# Autodesk Inventor assembly: Сборка1
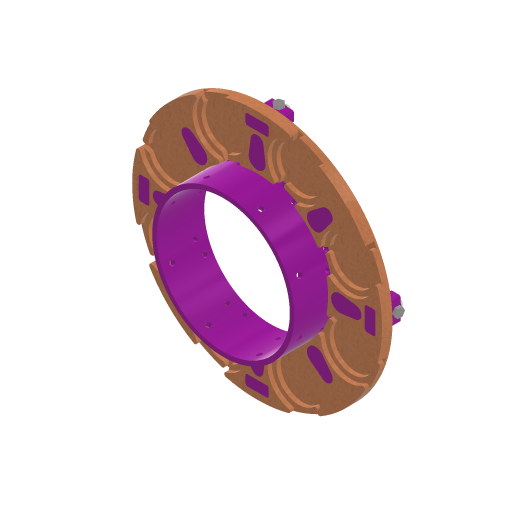
[picture p0: Inventor's stored thumbnail of the model, 512x512]
Saved by Autodesk Inventor 2023 (Build 270158000, 158)
## iProperties
Created: 2023-03-21
Part Number: Сборка1
Document SubType Name: Assembly
Designer: Admin
Author: Admin
## Documents named in this file (9)
- C:\Users\aleks\OneDrive\Рабочий стол\Хроматографический сортировщик\Детали\Хроматографичекий сортировщик.iam
- C:\Users\aleks\OneDrive\Рабочий стол\Хроматографический сортировщик\Детали\Барабан.ipt
- C:\Users\aleks\OneDrive\Рабочий стол\Хроматографический сортировщик\Детали\Покупные\Подшипник.ipt
- C:\Users\aleks\OneDrive\Рабочий стол\Хроматографический сортировщик\Детали\Покупные\Болт М5.ipt
- C:\Users\aleks\OneDrive\Рабочий стол\Хроматографический сортировщик\Детали\Покупные\Гайка М5 стопорная.ipt
- C:\Users\aleks\OneDrive\Рабочий стол\Хроматографический сортировщик\Детали\Покупные\Магнит.ipt
- C:\Users\aleks\OneDrive\Рабочий стол\Хроматографический сортировщик\Детали\Капсуль.ipt
- C:\Users\aleks\OneDrive\Рабочий стол\Хроматографический сортировщик\Детали\Покупные\Болт М5 круглый.ipt
- C:\Users\aleks\OneDrive\Рабочий стол\Хроматографический сортировщик\Детали\Короб для подшипника 2.0.ipt
## Components (49 placed, 8 different names)
1. Барабан:1 — Совмещение:57, Совмещение:58, Заподлицо:13, Совмещение:62, Совмещение:63, Совмещение:68, Совмещение:69, Заподлицо:15, Совмещение:70, Совмещение:71, Совмещение:76, Совмещение:77, Заподлицо:16, Совмещение:78, Совмещение:79, Заподлицо:17, Совмещение:84, Совмещение:85, Совмещение:102, Заподлицо:18, Совмещение:103, Совмещение:104, Заподлицо:19, Совмещение:105, Совмещение:106, Совмещение:107, Заподлицо:20, Совмещение:108, Совмещение:109, Заподлицо:21, Совмещение:111, Совмещение:112, Совмещение:113, Совмещение:114, Совмещение:115, Совмещение:116, Совмещение:117, Совмещение:118, Совмещение:119, Заподлицо:22, Совмещение:126, Совмещение:127, Заподлицо:23, Совмещение:134, Совмещение:135, Заподлицо:24, Совмещение:142, Совмещение:143, Заподлицо:25, Совмещение:150, Совмещение:151
2. Подшипник:1 — Совмещение:136, Совмещение:141
3. Подшипник:2 — Совмещение:128, Совмещение:131
4. Подшипник:3 — Совмещение:121, Совмещение:124
5. Подшипник:4 — Совмещение:145, Совмещение:146, Совмещение:148
6. Болт М5:1 — Совмещение:128, Совмещение:129, Совмещение:130, Совмещение:133
7. Гайка М5 стопорная:1 — Совмещение:129, Совмещение:132
8. Болт М5:2 — Совмещение:136, Совмещение:137, Совмещение:138, Совмещение:140
9. Гайка М5 стопорная:2 — Совмещение:137, Совмещение:139
10. Болт М5:3 — Совмещение:144, Совмещение:146, Совмещение:149
11. Гайка М5 стопорная:3 — Совмещение:122, Совмещение:123
12. Болт М5:4 — Совмещение:120, Совмещение:121, Совмещение:125
13. Гайка М5 стопорная:4 — Совмещение:145, Совмещение:147
14. Магнит:1 — Совмещение:94, Совмещение:95
15. Магнит:2 — Совмещение:66, Совмещение:67
16. Магнит:3 — Совмещение:59, Заподлицо:14
17. Магнит:4 — Совмещение:88, Совмещение:89
18. Магнит:5 — Совмещение:90, Совмещение:91
19. Магнит:6 — Совмещение:82, Совмещение:83
20. Магнит:7 — Совмещение:100, Совмещение:101
21. Магнит:8 — Совмещение:72, Совмещение:73
22. Капсуль:1 — Совмещение:57, Совмещение:58, Заподлицо:13, Совмещение:59, Заподлицо:14, Совмещение:60, Совмещение:61, Угол:1
23. Гайка М5 стопорная:5 — Совмещение:60, Совмещение:61, Угол:1
24. Болт М5 круглый:1 — Совмещение:62, Совмещение:63
25. Капсуль:2 — Совмещение:64, Угол:2, Совмещение:65, Совмещение:66, Совмещение:67, Совмещение:68, Совмещение:69, Заподлицо:15
26. Капсуль:3 — Совмещение:90, Совмещение:91, Совмещение:92, Угол:6, Совмещение:93, Совмещение:108, Совмещение:109, Заподлицо:21
27. Капсуль:4 — Совмещение:72, Совмещение:73, Совмещение:74, Угол:3, Совмещение:75, Совмещение:76, Совмещение:77, Заподлицо:16
28. Капсуль:5 — Совмещение:80, Угол:4, Совмещение:81, Совмещение:82, Совмещение:83, Заподлицо:17, Совмещение:84, Совмещение:85
29. Капсуль:6 — Совмещение:86, Угол:5, Совмещение:87, Совмещение:88, Совмещение:89, Совмещение:102, Заподлицо:18, Совмещение:103
30. Капсуль:7 — Совмещение:94, Совмещение:95, Совмещение:96, Угол:7, Совмещение:97, Совмещение:104, Заподлицо:19, Совмещение:105
31. Капсуль:8 — Совмещение:98, Угол:8, Совмещение:99, Совмещение:100, Совмещение:101, Совмещение:106, Совмещение:107, Заподлицо:20
32. Болт М5 круглый:2 — Совмещение:114, Совмещение:115
33. Гайка М5 стопорная:6 — Совмещение:98, Угол:8, Совмещение:99
34. Болт М5 круглый:3 — Совмещение:112, Совмещение:113
35. Гайка М5 стопорная:7 — Совмещение:96, Угол:7, Совмещение:97
36. Болт М5 круглый:4 — Совмещение:78, Совмещение:79
37. Гайка М5 стопорная:8 — Совмещение:86, Угол:5, Совмещение:87, Совмещение:110
38. Болт М5 круглый:5 — Совмещение:118, Совмещение:119
39. Гайка М5 стопорная:9 — Совмещение:80, Угол:4, Совмещение:81
40. Болт М5 круглый:6 — Совмещение:110, Совмещение:111
41. Гайка М5 стопорная:10 — Совмещение:92, Угол:6, Совмещение:93
42. Болт М5 круглый:7 — Совмещение:116, Совмещение:117
43. Гайка М5 стопорная:11 — Совмещение:74, Угол:3, Совмещение:75
44. Болт М5 круглый:8 — Совмещение:70, Совмещение:71
45. Гайка М5 стопорная:12 — Совмещение:64, Угол:2, Совмещение:65
46. Короб для подшипника 2.0:1 — Заподлицо:22, Совмещение:120, Совмещение:122, Совмещение:123, Совмещение:124, Совмещение:125, Совмещение:126, Совмещение:127
47. Короб для подшипника 2.0:2 — Заподлицо:23, Совмещение:130, Совмещение:131, Совмещение:132, Совмещение:133, Совмещение:134, Совмещение:135
48. Короб для подшипника 2.0:3 — Заподлицо:25, Совмещение:144, Совмещение:147, Совмещение:148, Совмещение:149, Совмещение:150, Совмещение:151
49. Короб для подшипника 2.0:4 — Совмещение:138, Совмещение:139, Совмещение:140, Совмещение:141, Заподлицо:24, Совмещение:142, Совмещение:143
## Relationships (116: Mate 95, Flush 13, Angle 8)
- Совмещение:57 [Mate]: Барабан:1 ↔ Капсуль:1
- Совмещение:58 [Mate]: Барабан:1 ↔ Капсуль:1
- Заподлицо:13 [Flush]: Барабан:1 ↔ Капсуль:1
- Совмещение:59 [Mate]: Магнит:3 ↔ Капсуль:1
- Заподлицо:14 [Flush]: Магнит:3 ↔ Капсуль:1
- Совмещение:60 [Mate]: Капсуль:1 ↔ Гайка М5 стопорная:5
- Совмещение:61 [Mate]: Капсуль:1 ↔ Гайка М5 стопорная:5
- Угол:1 [Angle] (0 deg): Капсуль:1 ↔ Гайка М5 стопорная:5
- Совмещение:62 [Mate]: Барабан:1 ↔ Болт М5 круглый:1
- Совмещение:63 [Mate]: Барабан:1 ↔ Болт М5 круглый:1
- Совмещение:64 [Mate]: Капсуль:2 ↔ Гайка М5 стопорная:12
- Угол:2 [Angle] (0 deg): Капсуль:2 ↔ Гайка М5 стопорная:12
- Совмещение:65 [Mate]: Капсуль:2 ↔ Гайка М5 стопорная:12
- Совмещение:66 [Mate]: Магнит:2 ↔ Капсуль:2
- Совмещение:67 [Mate]: Магнит:2 ↔ Капсуль:2
- Совмещение:68 [Mate]: Барабан:1 ↔ Капсуль:2
- Совмещение:69 [Mate]: Барабан:1 ↔ Капсуль:2
- Заподлицо:15 [Flush]: Барабан:1 ↔ Капсуль:2
- Совмещение:70 [Mate]: Барабан:1 ↔ Болт М5 круглый:8
- Совмещение:71 [Mate]: Барабан:1 ↔ Болт М5 круглый:8
- Совмещение:72 [Mate]: Магнит:8 ↔ Капсуль:4
- Совмещение:73 [Mate]: Магнит:8 ↔ Капсуль:4
- Совмещение:74 [Mate]: Капсуль:4 ↔ Гайка М5 стопорная:11
- Угол:3 [Angle] (0 deg): Капсуль:4 ↔ Гайка М5 стопорная:11
- Совмещение:75 [Mate]: Капсуль:4 ↔ Гайка М5 стопорная:11
- Совмещение:76 [Mate]: Барабан:1 ↔ Капсуль:4
- Совмещение:77 [Mate]: Барабан:1 ↔ Капсуль:4
- Заподлицо:16 [Flush]: Барабан:1 ↔ Капсуль:4
- Совмещение:78 [Mate]: Барабан:1 ↔ Болт М5 круглый:4
- Совмещение:79 [Mate]: Барабан:1 ↔ Болт М5 круглый:4
- Совмещение:80 [Mate]: Капсуль:5 ↔ Гайка М5 стопорная:9
- Угол:4 [Angle] (0 deg): Капсуль:5 ↔ Гайка М5 стопорная:9
- Совмещение:81 [Mate]: Капсуль:5 ↔ Гайка М5 стопорная:9
- Совмещение:82 [Mate]: Магнит:6 ↔ Капсуль:5
- Совмещение:83 [Mate]: Магнит:6 ↔ Капсуль:5
- Заподлицо:17 [Flush]: Барабан:1 ↔ Капсуль:5
- Совмещение:84 [Mate]: Барабан:1 ↔ Капсуль:5
- Совмещение:85 [Mate]: Барабан:1 ↔ Капсуль:5
- Совмещение:86 [Mate]: Капсуль:6 ↔ Гайка М5 стопорная:8
- Угол:5 [Angle] (0 deg): Капсуль:6 ↔ Гайка М5 стопорная:8
- Совмещение:87 [Mate]: Капсуль:6 ↔ Гайка М5 стопорная:8
- Совмещение:88 [Mate]: Магнит:4 ↔ Капсуль:6
- Совмещение:89 [Mate]: Магнит:4 ↔ Капсуль:6
- Совмещение:90 [Mate]: Магнит:5 ↔ Капсуль:3
- Совмещение:91 [Mate]: Магнит:5 ↔ Капсуль:3
- Совмещение:92 [Mate]: Капсуль:3 ↔ Гайка М5 стопорная:10
- Угол:6 [Angle] (0 deg): Капсуль:3 ↔ Гайка М5 стопорная:10
- Совмещение:93 [Mate]: Капсуль:3 ↔ Гайка М5 стопорная:10
- Совмещение:94 [Mate]: Магнит:1 ↔ Капсуль:7
- Совмещение:95 [Mate]: Магнит:1 ↔ Капсуль:7
- Совмещение:96 [Mate]: Капсуль:7 ↔ Гайка М5 стопорная:7
- Угол:7 [Angle] (0 deg): Капсуль:7 ↔ Гайка М5 стопорная:7
- Совмещение:97 [Mate]: Капсуль:7 ↔ Гайка М5 стопорная:7
- Совмещение:98 [Mate]: Капсуль:8 ↔ Гайка М5 стопорная:6
- Угол:8 [Angle] (0 deg): Капсуль:8 ↔ Гайка М5 стопорная:6
- Совмещение:99 [Mate]: Капсуль:8 ↔ Гайка М5 стопорная:6
- Совмещение:100 [Mate]: Магнит:7 ↔ Капсуль:8
- Совмещение:101 [Mate]: Магнит:7 ↔ Капсуль:8
- Совмещение:102 [Mate]: Барабан:1 ↔ Капсуль:6
- Заподлицо:18 [Flush]: Барабан:1 ↔ Капсуль:6
- Совмещение:103 [Mate]: Барабан:1 ↔ Капсуль:6
- Совмещение:104 [Mate]: Барабан:1 ↔ Капсуль:7
- Заподлицо:19 [Flush]: Барабан:1 ↔ Капсуль:7
- Совмещение:105 [Mate]: Барабан:1 ↔ Капсуль:7
- Совмещение:106 [Mate]: Барабан:1 ↔ Капсуль:8
- Совмещение:107 [Mate]: Барабан:1 ↔ Капсуль:8
- Заподлицо:20 [Flush]: Барабан:1 ↔ Капсуль:8
- Совмещение:108 [Mate]: Барабан:1 ↔ Капсуль:3
- Совмещение:109 [Mate]: Барабан:1 ↔ Капсуль:3
- Заподлицо:21 [Flush]: Барабан:1 ↔ Капсуль:3
- Совмещение:110 [Mate]: Гайка М5 стопорная:8 ↔ Болт М5 круглый:6
- Совмещение:111 [Mate]: Барабан:1 ↔ Болт М5 круглый:6
- Совмещение:112 [Mate]: Барабан:1 ↔ Болт М5 круглый:3
- Совмещение:113 [Mate]: Барабан:1 ↔ Болт М5 круглый:3
- Совмещение:114 [Mate]: Барабан:1 ↔ Болт М5 круглый:2
- Совмещение:115 [Mate]: Барабан:1 ↔ Болт М5 круглый:2
- Совмещение:116 [Mate]: Барабан:1 ↔ Болт М5 круглый:7
- Совмещение:117 [Mate]: Барабан:1 ↔ Болт М5 круглый:7
- Совмещение:118 [Mate]: Барабан:1 ↔ Болт М5 круглый:5
- Совмещение:119 [Mate]: Барабан:1 ↔ Болт М5 круглый:5
- Заподлицо:22 [Flush]: Барабан:1 ↔ Короб для подшипника 2.0:1
- Совмещение:120 [Mate]: Болт М5:4 ↔ Короб для подшипника 2.0:1
- Совмещение:121 [Mate]: Подшипник:3 ↔ Болт М5:4
- Совмещение:122 [Mate]: Гайка М5 стопорная:3 ↔ Короб для подшипника 2.0:1
- Совмещение:123 [Mate]: Гайка М5 стопорная:3 ↔ Короб для подшипника 2.0:1
- Совмещение:124 [Mate] (0.5 mm): Подшипник:3 ↔ Короб для подшипника 2.0:1
- Совмещение:125 [Mate]: Болт М5:4 ↔ Короб для подшипника 2.0:1
- Совмещение:126 [Mate]: Барабан:1 ↔ Короб для подшипника 2.0:1
- Совмещение:127 [Mate]: Барабан:1 ↔ Короб для подшипника 2.0:1
- Заподлицо:23 [Flush]: Барабан:1 ↔ Короб для подшипника 2.0:2
- Совмещение:128 [Mate]: Подшипник:2 ↔ Болт М5:1
- Совмещение:129 [Mate]: Болт М5:1 ↔ Гайка М5 стопорная:1
- Совмещение:130 [Mate]: Болт М5:1 ↔ Короб для подшипника 2.0:2
- Совмещение:131 [Mate] (0.5 mm): Подшипник:2 ↔ Короб для подшипника 2.0:2
- Совмещение:132 [Mate]: Гайка М5 стопорная:1 ↔ Короб для подшипника 2.0:2
- Совмещение:133 [Mate]: Болт М5:1 ↔ Короб для подшипника 2.0:2
- Совмещение:134 [Mate]: Барабан:1 ↔ Короб для подшипника 2.0:2
- Совмещение:135 [Mate]: Барабан:1 ↔ Короб для подшипника 2.0:2
- Совмещение:136 [Mate]: Подшипник:1 ↔ Болт М5:2
- Совмещение:137 [Mate]: Болт М5:2 ↔ Гайка М5 стопорная:2
- Совмещение:138 [Mate]: Болт М5:2 ↔ Короб для подшипника 2.0:4
- Совмещение:139 [Mate]: Гайка М5 стопорная:2 ↔ Короб для подшипника 2.0:4
- Совмещение:140 [Mate]: Болт М5:2 ↔ Короб для подшипника 2.0:4
- Совмещение:141 [Mate] (0.5 mm): Подшипник:1 ↔ Короб для подшипника 2.0:4
- Заподлицо:24 [Flush]: Барабан:1 ↔ Короб для подшипника 2.0:4
- Совмещение:142 [Mate]: Барабан:1 ↔ Короб для подшипника 2.0:4
- Совмещение:143 [Mate]: Барабан:1 ↔ Короб для подшипника 2.0:4
- Заподлицо:25 [Flush]: Барабан:1 ↔ Короб для подшипника 2.0:3
- Совмещение:144 [Mate]: Болт М5:3 ↔ Короб для подшипника 2.0:3
- Совмещение:145 [Mate]: Подшипник:4 ↔ Гайка М5 стопорная:4
- Совмещение:146 [Mate]: Подшипник:4 ↔ Болт М5:3
- Совмещение:147 [Mate]: Гайка М5 стопорная:4 ↔ Короб для подшипника 2.0:3
- Совмещение:148 [Mate] (0.5 mm): Подшипник:4 ↔ Короб для подшипника 2.0:3
- Совмещение:149 [Mate]: Болт М5:3 ↔ Короб для подшипника 2.0:3
- Совмещение:150 [Mate]: Барабан:1 ↔ Короб для подшипника 2.0:3
- Совмещение:151 [Mate]: Барабан:1 ↔ Короб для подшипника 2.0:3
